# Autodesk Inventor assembly: TVC Mount
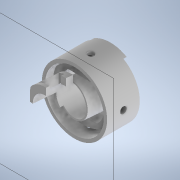
[picture p0: Inventor's stored thumbnail of the model, 180x180]
Saved by Autodesk Inventor 2022 (Build 260153000, 153)
## iProperties
Created: 2021-09-22
Part Number: TVC Mount
Document SubType Name: Assembly
Designer: WASHINGTON
Author: WASHINGTON
## Documents named in this file (5)
- D:\Thrust Vector Control\Thrust-Vector-Control\CAD\V2\TVC Mount.iam
- D:\Thrust Vector Control\Thrust-Vector-Control\CAD\V2\Part3.ipt
- D:\Thrust Vector Control\Thrust-Vector-Control\CAD\V2\Part1.ipt
- D:\Thrust Vector Control\Thrust-Vector-Control\CAD\V2\bolt.ipt
- D:\Thrust Vector Control\Thrust-Vector-Control\CAD\V2\aiirframe.ipt
## Components (5 placed, 4 different names)
1. Part3:1 — Mate:1, Mate:2, Rotation/Translation:1, Mate:3, Mate:4, Mate:5, Rotational:1, Cylindrical:1, Rotational:2, Mate:6, Mate:7
2. Part1:1 — Mate:1, Mate:2, Rotation/Translation:1, Rigid:1, Cylindrical:2
3. bolt:1 — Mate:3, Mate:4, Mate:5, Rotational:1, Rigid:1
4. bolt:2 — Cylindrical:1, Cylindrical:2, Rotational:2
5. aiirframe:2 — Mate:6, Mate:7
## Relationships (13: Mate 7, RevoluteJoint 2, CylindricalJoint 2, RelateRotateTranslate 1, WeldJoint 1)
- Mate:1: Part3:1 ↔ Part1:1
- Mate:2: Part3:1 ↔ Part1:1
- Rotation/Translation:1 [RelateRotateTranslate]: Part3:1 ↔ Part1:1
- Mate:3: Part3:1 ↔ bolt:1
- Mate:4: Part3:1 ↔ bolt:1
- Mate:5: Part3:1 ↔ bolt:1
- Rotational:1 [RevoluteJoint]: Part3:1 ↔ bolt:1
- Rigid:1 [WeldJoint]: Part1:1 ↔ bolt:1
- Cylindrical:1: Part3:1 ↔ bolt:2
- Cylindrical:2: Part1:1 ↔ bolt:2
- Rotational:2 [RevoluteJoint]: Part3:1 ↔ bolt:2
- Mate:6: Part3:1 ↔ aiirframe:2
- Mate:7: Part3:1 ↔ aiirframe:2
